# Autodesk Inventor assembly: 1110 ASY GBK long wall shield 1
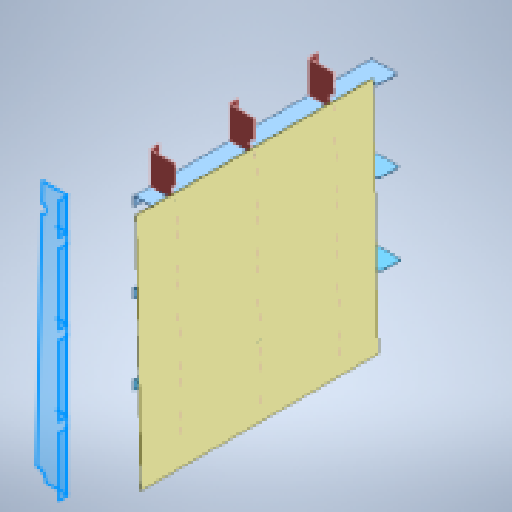
[picture p0: Inventor's stored thumbnail of the model, 512x512]
Saved by Autodesk Inventor 2026.2 (Build 302298000, 298)
## iProperties
Created: 2026-05-07
Part Number: 1110 ASY GBK long wall shield 1
Document SubType Name: Assembly
Designer: admin
Mass: 136093 g
Surface Area: 87957.2 cm^2
Volume: 17336.7 cm^3
Density: 7.85 g/cm^3
Author: admin
## Documents named in this file (6)
- C:\Users\admin\Documents\Inventor\GBK-Gubkinskiy\01 ASY GBK wall shield 1.1.1.iam
- C:\Users\admin\Documents\Inventor\GBK-Gubkinskiy\1019 GBK shield.ipt
- C:\Users\admin\Documents\Inventor\GBK-Gubkinskiy\GBK 1111 main rib.ipt
- C:\Users\admin\Documents\Inventor\GBK-Gubkinskiy\GBK 1112 stringer 1.ipt
- C:\Users\admin\Documents\Inventor\GBK-Gubkinskiy\GBK 1113 stringer 2.ipt
- C:\Users\admin\Documents\Inventor\GBK-Gubkinskiy\GBK 1114 stringer 3.ipt
## Components (7 placed, 6 different names)
1. 01.1 GBK shield.ipt:1 — Flush:5
2. 01.2 GBK main rib.ipt:1 — Rigid:1, Rigid:2, Rigid:3, Mate:3, Mate:5
3. 0234 GBK stringer 1:1 — Rigid:1, Rigid:4, Rigid:5
4. 0235 GBK stringer 2:1 — Rigid:2
5. 0236 GBK stringer 3:1 — Rigid:3
6. 01.2 GBK main rib:2 — Rigid:4
7. 01.2 GBK main rib:3 — Rigid:5
## Relationships (11: WeldJoint 5, Mate 4, Flush 2)
- [Mate]: 01.1 GBK shield.ipt:1 ↔ 01.2 GBK main rib.ipt:1
- [Flush] (254 mm): 01.1 GBK shield.ipt:1 ↔ 01.2 GBK main rib.ipt:1
- [Mate]: 01.1 GBK shield.ipt:1 ↔ 01.2 GBK main rib.ipt:1
- Rigid:1 [WeldJoint] (4 mm): 01.2 GBK main rib.ipt:1 ↔ 0234 GBK stringer 1:1
- Rigid:2 [WeldJoint] (4 mm): 01.2 GBK main rib.ipt:1 ↔ 0235 GBK stringer 2:1
- Rigid:3 [WeldJoint] (4 mm): 01.2 GBK main rib.ipt:1 ↔ 0236 GBK stringer 3:1
- Mate:3: 01.2 GBK main rib.ipt:1
- Flush:5: 01.1 GBK shield.ipt:1
- Mate:5: 01.2 GBK main rib.ipt:1
- Rigid:4 [WeldJoint] (4 mm): 0234 GBK stringer 1:1 ↔ 01.2 GBK main rib:2
- Rigid:5 [WeldJoint] (4 mm): 0234 GBK stringer 1:1 ↔ 01.2 GBK main rib:3
